# Autodesk Inventor assembly: 208_lc_resolver
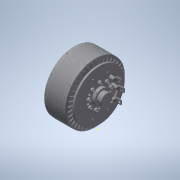
[picture p0: Inventor's stored thumbnail of the model, 180x180]
Saved by Autodesk Inventor 2021 (Build 250183000, 183)
## iProperties
Created: 2018-07-17
Part Number: 208_lc_resolver
Description: STEP AP203
Document SubType Name: Assembly
Designer: dandreal
Sending System: SolidWorks 2016
Preprocessor: SwSTEP 2.0
Title: 208_lc_resolver.STEP
Revision Number: ANY
## Documents named in this file (16)
- D:\PhotonUser\Downloads\Assembly Files-20201019T222523Z-001\Assembly Files\208_lc_resolver.iam
- D:\PhotonUser\Downloads\Assembly Files-20201019T222523Z-001\Assembly Files\stator_lc_cc_ass_208.iam
- D:\PhotonUser\Downloads\Assembly Files-20201019T222523Z-001\Assembly Files\rotor_assembly_lc_208.iam
- D:\PhotonUser\Downloads\Assembly Files-20201019T222523Z-001\Assembly Files\bearing_6206.ipt
- D:\PhotonUser\Downloads\Assembly Files-20201019T222523Z-001\Assembly Files\nut_lock_km6_m30x1,5.ipt
- D:\PhotonUser\Downloads\Assembly Files-20201019T222523Z-001\Assembly Files\washer_lock_mb6.ipt
- D:\PhotonUser\Downloads\Assembly Files-20201019T222523Z-001\Assembly Files\bracket_resolver_208_228.ipt
- D:\PhotonUser\Downloads\Assembly Files-20201019T222523Z-001\Assembly Files\shaft_res_enc_alu_208_228.ipt
- D:\PhotonUser\Downloads\Assembly Files-20201019T222523Z-001\Assembly Files\bolt_turned_imbus_m8x16.ipt
- D:\PhotonUser\Downloads\Assembly Files-20201019T222523Z-001\Assembly Files\spacer_outer_bearings_208_228.ipt
- D:\PhotonUser\Downloads\Assembly Files-20201019T222523Z-001\Assembly Files\Bracket_X_208.ipt
- D:\PhotonUser\Downloads\Assembly Files-20201019T222523Z-001\Assembly Files\bolt_imbus_m8x30.ipt
- D:\PhotonUser\Downloads\Assembly Files-20201019T222523Z-001\Assembly Files\ring_sealing_assembly_208_228_268.ipt
- D:\PhotonUser\Downloads\Assembly Files-20201019T222523Z-001\Assembly Files\ring_sliding_ssteel_208_228_268.ipt
- D:\PhotonUser\Downloads\Assembly Files-20201019T222523Z-001\Assembly Files\resolver_1pp.ipt
- D:\PhotonUser\Downloads\Assembly Files-20201019T222523Z-001\Assembly Files\cover_res1.ipt
## Components (24 placed, 24 different names)
1. stator_lc_cc_ass_208_1 [sub-assembly]
2. rotor_assembly_lc_208_2 [sub-assembly]
3. bearing_6206_3
4. nut_lock_km6_m30x1,5_4
5. washer_lock_mb6_5
6. bracket_resolver_208_228_6 — Insert:1
7. shaft_res_enc_alu_208_228_7
8. bolt_turned_imbus_m8x16_8
9. bearing_6206_9
10. spacer_outer_bearings_208_228_10
11. bolt_imbus_m8x30_12
12. bolt_imbus_m8x30_13
13. bolt_imbus_m8x30_14
14. bolt_imbus_m8x30_15
15. bolt_imbus_m8x30_16
16. bolt_imbus_m8x30_17
17. bolt_imbus_m8x30_18
18. bolt_imbus_m8x30_19
19. bolt_imbus_m8x30_20
20. ring_sealing_assembly_208_228_268_21
21. ring_sliding_ssteel_208_228_268_22
22. resolver_1pp_23
23. cover_res1_24
24. Bracket_X_208:1 — Insert:1
## Relationships (1: Insert 1)
- Insert:1: bracket_resolver_208_228_6 ↔ Bracket_X_208:1
